# Autodesk Inventor assembly: CableBraider
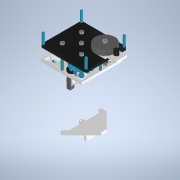
[picture p0: Inventor's stored thumbnail of the model, 180x180]
Saved by Autodesk Inventor 2021 (Build 250183000, 183)
## iProperties
Created: 2020-07-21
Part Number: CableBraider
Document SubType Name: Assembly
Designer: elmar
Author: elmar
## Documents named in this file (15)
- D:\FourWireBraidingMachine\InventorFiles\CableBraider.iam
- D:\FourWireBraidingMachine\InventorFiles\BasePlate.ipt
- D:\FourWireBraidingMachine\InventorFiles\DriveGear.ipt
- D:\FourWireBraidingMachine\InventorFiles\HornGear.ipt
- D:\FourWireBraidingMachine\InventorFiles\Standoff.ipt
- D:\FourWireBraidingMachine\InventorFiles\GuidePlateV1.ipt
- D:\FourWireBraidingMachine\InventorFiles\ReductionGearBracket.ipt
- D:\FourWireBraidingMachine\InventorFiles\ReductionGear.ipt
- D:\FourWireBraidingMachine\InventorFiles\ReductionDriveGear.ipt
- D:\FourWireBraidingMachine\InventorFiles\HornGearMirror.ipt
- D:\FourWireBraidingMachine\InventorFiles\WinderAssembly.iam
- C:\Users\elmar\OneDrive\Documents\Inventor\Content Center Files\R2021\en-US\ANSI B18.2.4.2M\ANSI B18.2.4.2M - M8x1.25 - 13.ipt
- D:\FourWireBraidingMachine\InventorFiles\Carriage.iam
- C:\Users\elmar\OneDrive\Documents\Inventor\Content Center Files\R2021\en-US\AS 1237 (2.1)\AS 1237 - 8.ipt
- C:\Users\elmar\OneDrive\Documents\Inventor\Content Center Files\R2021\en-US\AS 1112 (2)\AS 1112 - M8  Type 5.ipt
## Components (33 placed, 14 different names)
1. BasePlate:1 — Mate:1, Mate:2, Mate:3, Insert:3, Insert:5, Angle:1, Insert:15, Insert:17, Insert:18, Insert:19, Insert:20, Insert:21, Insert:22, Insert:23, Insert:24, Insert:25, Insert:26, Insert:28, Insert:31, Insert:38
2. DriveGear:1 — Insert:31, Insert:34
3. HornGear:1 — Insert:3
4. Standoff:1 — Insert:5
5. GuidePlateV1:1 — Mate:4, Insert:29, Insert:30, Insert:37, Mate:5
6. ReductionGearBracket:1 — Angle:1, Insert:12, Insert:15, Insert:33
7. ReductionDriveGear:1 — Insert:12
8. ReductionGear:1 — Insert:33, Insert:36
9. Standoff:2 — Insert:17
10. HornGear:2 — Insert:18
11. HornGearMirror:1 — Insert:20
12. HornGearMirror:2 — Insert:19
13. Standoff:3 — Insert:21
14. Standoff:4 — Insert:23
15. Standoff:5 — Insert:25
16. Standoff:6 — Insert:22, Insert:29
17. Standoff:7 — Insert:24, Insert:30
18. Standoff:8 — Insert:26
19. WinderAssembly:1 [sub-assembly] — Insert:37, Mate:5
20. Carriage:1 [sub-assembly] — Mate:4
21. ANSI B18.2.4.2M M8x1.25:2 — Insert:35
22. AS 1237 (2.1) 8:1 — Insert:34, Insert:35
23. ANSI B18.2.4.2M M8x1.25:3 — Insert:36
24. ANSI B18.2.4.2M M8x1.25:1 — Insert:28
25. ANSI B18.2.4.2M M8x1.25:4
26. AS 1112 (2) - Metric M8  Type 5:1 — Insert:38
27. AS 1112 (2) - Metric M8  Type 5:2
28. AS 1112 (2) - Metric M8  Type 5:3
29. AS 1112 (2) - Metric M8  Type 5:4
30. AS 1112 (2) - Metric M8  Type 5:5
31. AS 1112 (2) - Metric M8  Type 5:6
32. AS 1112 (2) - Metric M8  Type 5:7
33. AS 1112 (2) - Metric M8  Type 5:8
## Component patterns: (2 elements, first: ANSI B18.2.4.2M M8x1.25:1), (4 elements, first: AS 1112 (2) - Metric M8  Type 5:1), Component Pattern 1:2 (4 elements)
## Relationships (30: Insert 24, Mate 5, Angle 1)
- Mate:1: BasePlate:1
- Mate:2: BasePlate:1
- Mate:3: BasePlate:1
- Insert:3 (1 mm): BasePlate:1 ↔ HornGear:1
- Insert:5: BasePlate:1 ↔ Standoff:1
- Angle:1 (0 deg): BasePlate:1 ↔ ReductionGearBracket:1
- Insert:12 (1 mm): ReductionGearBracket:1 ↔ ReductionDriveGear:1
- Insert:15: BasePlate:1 ↔ ReductionGearBracket:1
- Insert:17: BasePlate:1 ↔ Standoff:2
- Insert:18 (1 mm): BasePlate:1 ↔ HornGear:2
- Insert:19 (1 mm): BasePlate:1 ↔ HornGearMirror:2
- Insert:20 (1 mm): BasePlate:1 ↔ HornGearMirror:1
- Insert:21: BasePlate:1 ↔ Standoff:3
- Insert:22: BasePlate:1 ↔ Standoff:6
- Insert:23: BasePlate:1 ↔ Standoff:4
- Insert:24: BasePlate:1 ↔ Standoff:7
- Insert:25: BasePlate:1 ↔ Standoff:5
- Insert:26: BasePlate:1 ↔ Standoff:8
- Insert:28: BasePlate:1 ↔ ANSI B18.2.4.2M M8x1.25:1
- Mate:4: GuidePlateV1:1 ↔ Carriage:1
- Insert:29: GuidePlateV1:1 ↔ Standoff:6
- Insert:30: GuidePlateV1:1 ↔ Standoff:7
- Insert:31 (1 mm): BasePlate:1 ↔ DriveGear:1
- Insert:33 (1 mm): ReductionGearBracket:1 ↔ ReductionGear:1
- Insert:34: DriveGear:1 ↔ AS 1237 (2.1) 8:1
- Insert:35: ANSI B18.2.4.2M M8x1.25:2 ↔ AS 1237 (2.1) 8:1
- Insert:36: ReductionGear:1 ↔ ANSI B18.2.4.2M M8x1.25:3
- Insert:37 (200 mm): GuidePlateV1:1 ↔ WinderAssembly:1
- Mate:5: GuidePlateV1:1 ↔ WinderAssembly:1
- Insert:38: BasePlate:1 ↔ AS 1112 (2) - Metric M8  Type 5:1
